# Autodesk Inventor assembly: BallShooterV02
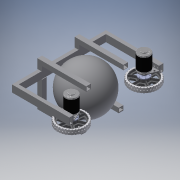
[picture p0: Inventor's stored thumbnail of the model, 180x180]
Saved by Autodesk Inventor 2016 SP1 (Build 200210100, 210)
## iProperties
Created: 2016-01-24
Part Number: BallShooterV02
Document SubType Name: Assembly
Designer: steele
Author: steele
## Documents named in this file (7)
- C:\snobotics\CAD-Development\robSteele\SnoBotics2016\2016-01-27-BallShooter\BallShooterV02.iam
- C:\snobotics\CAD-MfgResources\Andy-Mark\MotorMounts\AM 2488 CIM bracket.ipt
- C:\snobotics\CAD-MfgResources\Andy-Mark\Hubs\am-0320a_8mm_Key_Hub.ipt
- C:\snobotics\CAD-Development\robSteele\SnoBotics2016\DraftOfBoulder.ipt
- C:\snobotics\autodesk\2016\FRC KOP 2016\Motors\MOT_MiniCIMMotor_217-3371.ipt
- C:\snobotics\CAD-Development\robSteele\SnoBotics2016\2016-01-23-BallShooter\am-940a-6-HiGrip-.iam
- C:\snobotics\CAD-Development\robSteele\SnoBotics2016\2016-01-27-BallShooter\ShooterFrame.ipt
## Components (10 placed, 6 different names)
1. ShooterFrame:1 — Flush:3, Mate:7, Flush:4, Flush:5, Mate:8, Mate:9, Flush:6, Flush:7
2. AM 2488 CIM bracket:1 — Insert:4, Insert:6, Mate:9, Flush:6, Flush:7
3. MOT_MiniCIMMotor_217-3371:1 — Insert:4
4. am-0320a_8mm_Key_Hub:1 — Insert:5, Insert:6
5. am-940a-6-HiGrip-:1 [sub-assembly] — Insert:5, Mate:5
6. DraftOfBoulder:1 — Mate:5, Flush:3, Mate:8
7. AM 2488 CIM bracket:2 — Mate:7, Flush:4, Flush:5
8. am-0320a_8mm_Key_Hub:2
9. MOT_MiniCIMMotor_217-3371:2
10. am-940a-6-HiGrip-:2 [sub-assembly]
## Relationships (15: Insert 6, Flush 5, Mate 4)
- Insert:4: AM 2488 CIM bracket:1 ↔ MOT_MiniCIMMotor_217-3371:1
- Insert:5: am-0320a_8mm_Key_Hub:1 ↔ am-940a-6-HiGrip-:1
- Insert:6: AM 2488 CIM bracket:1 ↔ am-0320a_8mm_Key_Hub:1
- Mate:5: am-940a-6-HiGrip-:1 ↔ DraftOfBoulder:1
- Flush:3 (127 mm): ShooterFrame:1 ↔ DraftOfBoulder:1
- [Insert]: AM 2488 CIM bracket:2 ↔ MOT_MiniCIMMotor_217-3371:2
- [Insert]: am-0320a_8mm_Key_Hub:2 ↔ am-940a-6-HiGrip-:2
- [Insert]: AM 2488 CIM bracket:2 ↔ am-0320a_8mm_Key_Hub:2
- Mate:7: ShooterFrame:1 ↔ AM 2488 CIM bracket:2
- Flush:4: ShooterFrame:1 ↔ AM 2488 CIM bracket:2
- Flush:5: ShooterFrame:1 ↔ AM 2488 CIM bracket:2
- Mate:8: ShooterFrame:1 ↔ DraftOfBoulder:1
- Mate:9: ShooterFrame:1 ↔ AM 2488 CIM bracket:1
- Flush:6: ShooterFrame:1 ↔ AM 2488 CIM bracket:1
- Flush:7: ShooterFrame:1 ↔ AM 2488 CIM bracket:1
## Named parameters: d36_d19 = 0 mm, d37_d25 = 0 mm, d38_d26 = 0 mm
